# Autodesk Inventor assembly: WCP SS Flipped Gearbox (SingleSpeed, 2 Stages)
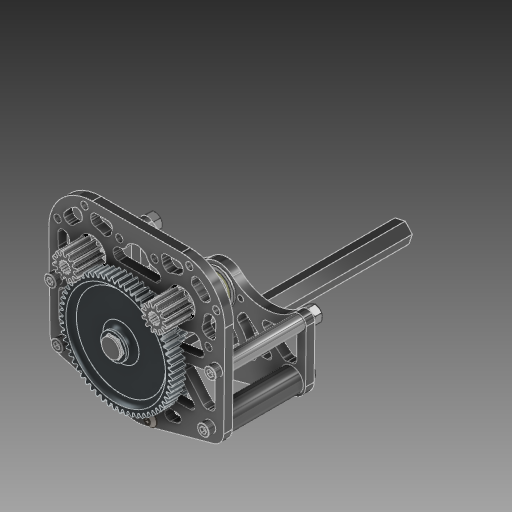
[picture p0: Inventor's stored thumbnail of the model, 512x512]
Saved by Autodesk Inventor 2023 (Build 270158030, 158C)
## iProperties
Created: 2019-12-21
Part Number: WCP SS Flipped Gearbox (SingleSpeed, 2 Stages)
Description: STEP AP214
Document SubType Name: Assembly
Designer: mkbos
Mass: 676.362 g
Surface Area: 1112.64 cm^2
Volume: 172.525 cm^3
Density: 3.92038 g/cm^3
Sending System: SolidWorks 2018
Preprocessor: SwSTEP 2.0
Title: WCP-0235 Rev1 - WCP SS Flipped Gearbox (SingleSpeed, 2 Stages).STEP
Revision Number: ANY
## Documents named in this file (24)
- D:\Collaborative Robots\COTS Parts\General Gearboxes\COTS Gearboxes\WCP Gearbox\WCP SS Flipped Gearbox (SingleSpeed, 2 Stages).iam
- D:\Collaborative Robots\COTS Parts\General Gearboxes\COTS Gearboxes\WCP Gearbox\WCP-0235-001 Rev1.ipt
- D:\Collaborative Robots\COTS Parts\General Gearboxes\COTS Gearboxes\WCP Gearbox\WCP-0235-002 Rev1.ipt
- D:\Collaborative Robots\COTS Parts\General Gearboxes\COTS Gearboxes\WCP Gearbox\BHCS_10-32_0_250_91255A261_91255A261.ipt
- D:\Collaborative Robots\COTS Parts\General Gearboxes\COTS Gearboxes\WCP Gearbox\WCP-0155-012 Rev1.ipt
- D:\Collaborative Robots\COTS Parts\General Gearboxes\COTS Gearboxes\WCP Gearbox\WCP-0235-003 Rev1.ipt
- D:\Collaborative Robots\COTS Parts\General Gearboxes\COTS Gearboxes\WCP Gearbox\WCP-0235-004 Rev1.ipt
- D:\Collaborative Robots\COTS Parts\Power Transfer\Bearings and Bushings\Bearings\FR6.ipt
- D:\FRC 1369 Minotaur\2020.5 Minotaur\Collaborative Parts Lib\Power Transfer\Bearings.ipt
- D:\Collaborative Robots\COTS Parts\Power Transfer\Bearings and Bushings\Bearings\FR8.ipt
- D:\FRC 1369 Minotaur\2020.5 Minotaur\Collaborative Parts Lib\Power Transfer\VexPro Spur Gears.ipt
- D:\Collaborative Robots\COTS Parts\Power Transfer\Depricated\Motor Output\Gears\Falcon 12T Pinion (VexPro #217-6919).ipt
- D:\Collaborative Robots\COTS Parts\Power Transfer\Gears (Hex)\Spur Gear2\20dp 22T VexPro 500 Hex Steel Gear.ipt
- D:\Collaborative Robots\COTS Parts\Power Transfer\Bearings and Bushings\Bearings\FR8 Hex.ipt
- D:\Collaborative Robots\COTS Parts\Power Transfer\Gears (Hex)\Spur Gear2\20dp 26T VexPro 500 Hex Steel Gear.ipt
- D:\Collaborative Robots\COTS Parts\Power Transfer\Gears (Hex)\Spur Gear2\20dp 60T VexPro 500 Hex Steel Gear (Pocketed).ipt
- D:\FRC 1369 Minotaur\2020.5 Minotaur\Collaborative Parts Lib\Hardware\Spacers & Standoffs.ipt
- D:\Collaborative Robots\COTS Parts\Hardware\Spacers\Spacers & Standoffs\VexPro 500 Hex Spacer 0.125in.ipt
- D:\Collaborative Robots\COTS Parts\Hardware\Spacers\Spacers & Standoffs\VexPro 500 Hex Spacer 0.0625in.ipt
- D:\Collaborative Robots\COTS Parts\Hardware\Spacers\Spacers & Standoffs\WCP Aluminum Standoff (No. 10 x 2Lg x 0.375OD).ipt
- D:\Collaborative Robots\COTS Parts\Hardware\Fasteners\Machine Screws\10-32 UNFx2.75 Socket Head Cap Screw.ipt
- D:\FRC 1369 Minotaur\2020.5 Minotaur\Collaborative Parts Lib\Hardware\Machine Screws.ipt
- D:\Collaborative Robots\COTS Parts\Hardware\Nuts and Threaded Blocks\Nuts\10-32 Regular Nylon locknut.ipt
- D:\FRC 1369 Minotaur\2020.5 Minotaur\Collaborative Parts Lib\Hardware\Nuts.ipt
## Components (28 placed, 20 different names)
1. WCP-0235-001 Rev1_1 — Insert:2, Insert:3, Insert:4, Insert:5, Insert:13, Insert:14, Insert:15, Insert:16, Insert:19, Insert:20
2. WCP-0235-002 Rev1_2 — Insert:1, Insert:17, Insert:18, Insert:21, Insert:22, Mate:5
3. BHCS_10-32_0_250_91255A261_91255A261_7
4. WCP-0155-012 Rev1_13 — Mate:1, Mate:2, Insert:7
5. WCP-0235-003 Rev1_15 — Insert:11, Mate:4, Insert:12
6. BHCS_10-32_0_250_91255A261_91255A261_18
7. WCP-0235-004 Rev1_21
8. WCP-0235-004 Rev1_22
9. FR6:1 — Insert:1, Insert:12
10. FR8:2 — Insert:2, Insert:7, Insert:10
11. Falcon 12T Pinion (VexPro #217-6919):1 — Insert:3
12. Falcon 12T Pinion (VexPro #217-6919):2 — Insert:4
13. 20dp 22T VexPro 500 Hex Steel Gear:1 — Insert:6
14. FR8 Hex:5 — Insert:5, Insert:6, Insert:8
15. 20dp 26T VexPro 500 Hex Steel Gear:2 — Mate:1, Mate:2, Mate:3
16. 20dp 60T VexPro 500 Hex Steel Gear (Pocketed):3 — Insert:9, Insert:11, Mate:4
17. VexPro 500 Hex Spacer 0.125in:2 — Insert:8, Insert:9
18. VexPro 500 Hex Spacer 0.0625in:3 — Insert:10, Mate:3
19. WCP Aluminum Standoff (No. 10 x 2Lg x 0.375OD):4 — Insert:13
20. WCP Aluminum Standoff (No. 10 x 2Lg x 0.375OD):5 — Insert:14
21. 10-32 UNFx2.75 Socket Head Cap Screw:1 — Insert:19
22. 10-32 UNFx2.75 Socket Head Cap Screw:2 — Insert:16
23. 10-32 UNFx2.75 Socket Head Cap Screw:3 — Insert:20
24. 10-32 UNFx2.75 Socket Head Cap Screw:4 — Insert:15, Mate:5
25. 10-32 Regular Nylon locknut:1 — Insert:17
26. 10-32 Regular Nylon locknut:2 — Insert:18
27. 10-32 Regular Nylon locknut:3 — Insert:21
28. 10-32 Regular Nylon locknut:4 — Insert:22
## Relationships (27: Insert 22, Mate 5)
- Insert:1: WCP-0235-002 Rev1_2 ↔ FR6:1
- Insert:2: WCP-0235-001 Rev1_1 ↔ FR8:2
- Insert:3: WCP-0235-001 Rev1_1 ↔ Falcon 12T Pinion (VexPro #217-6919):1
- Insert:4: WCP-0235-001 Rev1_1 ↔ Falcon 12T Pinion (VexPro #217-6919):2
- Insert:5: WCP-0235-001 Rev1_1 ↔ FR8 Hex:5
- Insert:6: 20dp 22T VexPro 500 Hex Steel Gear:1 ↔ FR8 Hex:5
- Mate:1: WCP-0155-012 Rev1_13 ↔ 20dp 26T VexPro 500 Hex Steel Gear:2
- Mate:2: WCP-0155-012 Rev1_13 ↔ 20dp 26T VexPro 500 Hex Steel Gear:2
- Insert:7: WCP-0155-012 Rev1_13 ↔ FR8:2
- Insert:8: FR8 Hex:5 ↔ VexPro 500 Hex Spacer 0.125in:2
- Insert:9: 20dp 60T VexPro 500 Hex Steel Gear (Pocketed):3 ↔ VexPro 500 Hex Spacer 0.125in:2
- Insert:10: FR8:2 ↔ VexPro 500 Hex Spacer 0.0625in:3
- Mate:3: 20dp 26T VexPro 500 Hex Steel Gear:2 ↔ VexPro 500 Hex Spacer 0.0625in:3
- Insert:11: WCP-0235-003 Rev1_15 ↔ 20dp 60T VexPro 500 Hex Steel Gear (Pocketed):3
- Mate:4: WCP-0235-003 Rev1_15 ↔ 20dp 60T VexPro 500 Hex Steel Gear (Pocketed):3
- Insert:12: WCP-0235-003 Rev1_15 ↔ FR6:1
- Insert:13: WCP-0235-001 Rev1_1 ↔ WCP Aluminum Standoff (No. 10 x 2Lg x 0.375OD):4
- Insert:14: WCP-0235-001 Rev1_1 ↔ WCP Aluminum Standoff (No. 10 x 2Lg x 0.375OD):5
- Insert:15: WCP-0235-001 Rev1_1 ↔ 10-32 UNFx2.75 Socket Head Cap Screw:4
- Insert:16: WCP-0235-001 Rev1_1 ↔ 10-32 UNFx2.75 Socket Head Cap Screw:2
- Insert:17: WCP-0235-002 Rev1_2 ↔ 10-32 Regular Nylon locknut:1
- Insert:18: WCP-0235-002 Rev1_2 ↔ 10-32 Regular Nylon locknut:2
- Insert:19: WCP-0235-001 Rev1_1 ↔ 10-32 UNFx2.75 Socket Head Cap Screw:1
- Insert:20: WCP-0235-001 Rev1_1 ↔ 10-32 UNFx2.75 Socket Head Cap Screw:3
- Insert:21: WCP-0235-002 Rev1_2 ↔ 10-32 Regular Nylon locknut:3
- Insert:22: WCP-0235-002 Rev1_2 ↔ 10-32 Regular Nylon locknut:4
- Mate:5: WCP-0235-002 Rev1_2 ↔ 10-32 UNFx2.75 Socket Head Cap Screw:4
